# Autodesk Inventor assembly: Assembly1
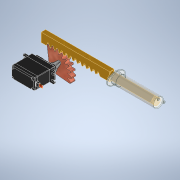
[picture p0: Inventor's stored thumbnail of the model, 180x180]
Saved by Autodesk Inventor 2022 (Build 260153000, 153)
## iProperties
Created: 2022-06-04
Part Number: Assembly1
Document SubType Name: Assembly
Designer: frede
Author: frede
## Documents named in this file (8)
- C:\Users\frede\OneDrive\Desktop\DigCow\Assembly1.iam
- C:\Users\frede\Downloads\Servo Motor MG996R.ipt
- C:\Users\frede\OneDrive\Desktop\Servo Motor MG996R - Copy.ipt
- C:\Users\frede\OneDrive\Desktop\DigCow\Rack222.ipt
- C:\Users\frede\OneDrive\Desktop\DigCow\Pinion222.ipt
- C:\Users\frede\OneDrive\Desktop\DigCow\Syringe.ipt
- C:\Users\frede\OneDrive\Desktop\DigCow\RackSlider.ipt
- C:\Users\frede\OneDrive\Documents\Inventor\Content Center Files\R2022\en-US\DIN 912\DIN 912 - M3 x 0.5 x 10 x 8.75.ipt
## Components (7 placed, 7 different names)
1. Servo Motor MG996R:1 — Rotational:1, Angle:2, Flush:2, Angle:3, Flush:3
2. Arm — Rotational:1, Insert:1, Angle:1
3. Rack222:1 — Flush:1, Angle:2, Flush:2, Rotation/Translation:1, Insert:2, Mate:1, Mate:2
4. Pinion222:1 — Insert:1, Angle:1, Flush:1, Rotation/Translation:1, Insert:3, Rotation:1
5. Syringe:1 — Insert:2, Angle:3
6. RackSlider:1 — Mate:1, Mate:2, Flush:3
7. DIN 912 - replaced by DIN EN ISO 4762 M3 x 10:1 — Insert:3, Rotation:1
## Relationships (14: Insert 3, Angle 3, Flush 3, Mate 2, RevoluteJoint 1, RelateRotateTranslate 1, RelateRotation 1)
- Rotational:1 [RevoluteJoint]: Servo Motor MG996R:1 ↔ Arm
- Insert:1: Arm ↔ Pinion222:1
- Angle:1 (0 deg): Arm ↔ Pinion222:1
- Flush:1: Rack222:1 ↔ Pinion222:1
- Angle:2 (0 deg): Servo Motor MG996R:1 ↔ Rack222:1
- Flush:2 (32.6 mm): Servo Motor MG996R:1 ↔ Rack222:1
- Rotation/Translation:1 [RelateRotateTranslate] (183 mm): Rack222:1 ↔ Pinion222:1
- Insert:2 (62.5 mm): Rack222:1 ↔ Syringe:1
- Angle:3 (0 deg): Servo Motor MG996R:1 ↔ Syringe:1
- Mate:1 (0.1 mm): Rack222:1 ↔ RackSlider:1
- Mate:2 (0.5 mm): Rack222:1 ↔ RackSlider:1
- Flush:3 (53 mm): Servo Motor MG996R:1 ↔ RackSlider:1
- Insert:3: Pinion222:1 ↔ DIN 912 - replaced by DIN EN ISO 4762 M3 x 10:1
- Rotation:1 [RelateRotation] (1 ul): Pinion222:1 ↔ DIN 912 - replaced by DIN EN ISO 4762 M3 x 10:1
